# Autodesk Inventor assembly: singleHookHangerV01
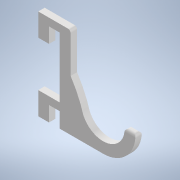
[picture p0: Inventor's stored thumbnail of the model, 180x180]
Saved by Autodesk Inventor 2020.2 (Build 242310000, 310)
## iProperties
Created: 2020-03-15
Part Number: singleHookHangerV01
Document SubType Name: Assembly
Designer: robst
Author: robst
## Documents named in this file (3)
- C:\git\CAD-Development\robSteele\HouseProjects\Garage\Ikea\singleHookHangerV01.iam
- C:\git\CAD-Development\robSteele\HouseProjects\Garage\Ikea\oneStartConfigurationV01.ipt
- C:\git\CAD-Development\robSteele\HouseProjects\Garage\Ikea\hook.ipt
## Components (2 placed, 2 different names)
1. oneStartConfigurationV01:1 — Mate:1, Flush:1, Flush:2
2. hook:1 — Mate:1, Flush:1, Flush:2
## Relationships (3: Flush 2, Mate 1)
- Mate:1: oneStartConfigurationV01:1 ↔ hook:1
- Flush:1: oneStartConfigurationV01:1 ↔ hook:1
- Flush:2: oneStartConfigurationV01:1 ↔ hook:1
